# Autodesk Inventor assembly: KB33-046-002 - Привод в сборе
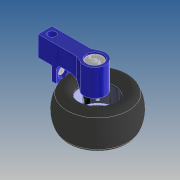
[picture p0: Inventor's stored thumbnail of the model, 180x180]
Saved by Autodesk Inventor 2020 (Build 240168000, 168)
## iProperties
Created: 2021-06-21
Part Number: KB33-046-002 - Привод в сборе
Document SubType Name: Assembly
Designer: Петров Иван
Mass: 1277.54 g
Surface Area: 1658.08 cm^2
Volume: 1247.52 cm^3
Density: 1.02407 g/cm^3
Author: Петров Иван
## Documents named in this file (6)
- E:\IVAN\Ivan_desktop\Kvantorium\Projects\RoboPatrol\design\KB33-046-002 - Привод в сборе.iam
- E:\IVAN\Ivan_desktop\Kvantorium\Projects\RoboPatrol\design\KB33-046-002-001 - Крепление.ipt
- E:\IVAN\Ivan_desktop\Kvantorium\Projects\RoboPatrol\design\standart_components\dc_gear_motor_12V_500rpm\dc_gear_motor_12V_500rpm.ipt
- E:\IVAN\Ivan_desktop\Kvantorium\Projects\RoboPatrol\design\standart_components\WheelBig\колесо большое1.iam
- C:\Users\Петров Иван\Documents\Inventor\Content Center Files\R2020\ru-RU\GOST 17475-80 (2)\Винт 2.M8-6gx16 ГОСТ 17475-80.ipt
- C:\Users\Петров Иван\Documents\Inventor\Content Center Files\R2020\ru-RU\GOST 17475-80 (2)\Винт 2.M8-6gx30 ГОСТ 17475-80.ipt
## Components (5 placed, 5 different names)
1. KB33-046-002-001 - Крепление:1 — Заподлицо:1, Совмещение:1, Совмещение:2, Вставка:2, Вставка:3
2. dc_gear_motor_12V_500rpm:1 — Заподлицо:1, Совмещение:1, Совмещение:2, Совмещение:3, Совмещение:4
3. колесо большое1:1 [sub-assembly] — Совмещение:3, Совмещение:4
4. Винт 2 ГОСТ 17475-80 M8 x 16:1 — Вставка:2
5. Винт 2 ГОСТ 17475-80 M8 x 30:1 — Вставка:3
## Relationships (7: Mate 4, Insert 2, Flush 1)
- Заподлицо:1 [Flush]: KB33-046-002-001 - Крепление:1 ↔ dc_gear_motor_12V_500rpm:1
- Совмещение:1 [Mate]: KB33-046-002-001 - Крепление:1 ↔ dc_gear_motor_12V_500rpm:1
- Совмещение:2 [Mate]: KB33-046-002-001 - Крепление:1 ↔ dc_gear_motor_12V_500rpm:1
- Совмещение:3 [Mate] (30 mm): dc_gear_motor_12V_500rpm:1 ↔ колесо большое1:1
- Совмещение:4 [Mate]: dc_gear_motor_12V_500rpm:1 ↔ колесо большое1:1
- Вставка:2 [Insert]: KB33-046-002-001 - Крепление:1 ↔ Винт 2 ГОСТ 17475-80 M8 x 16:1
- Вставка:3 [Insert]: KB33-046-002-001 - Крепление:1 ↔ Винт 2 ГОСТ 17475-80 M8 x 30:1
